# Autodesk Inventor assembly: Tensioner
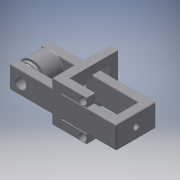
[picture p0: Inventor's stored thumbnail of the model, 180x180]
Saved by Autodesk Inventor 2017 (Build 210142000, 142)
## iProperties
Created: 2017-07-29
Part Number: Tensioner
Document SubType Name: Assembly
Designer: User
Author: User
## Documents named in this file (5)
- C:\Robotics\CAD\2016-17_CAD\DriveTrain\Tensioner.iam
- C:\Robotics\CAD\2016-17_CAD\DriveTrain\TensionerAxleHolder.ipt
- C:\Robotics\CAD\2016-17_CAD\DriveTrain\TensionerPlate.ipt
- C:\Robotics\CAD\COTSParts\Bearings - AndyMark\Bearing 250 ID 500 OD flanged_MIR.ipt
- C:\Robotics\CAD\2016-17_CAD\Custom COTS\Spacer.5inBore.378Width.ipt
## Components (5 placed, 4 different names)
1. TensionerAxleHolder:1 — Mate:1, Flush:1, Flush:2, Insert:3, Insert:4
2. TensionerPlate:1 — Mate:1, Flush:1, Flush:2
3. Bearing 250 ID 500 OD flanged_MIR:1 — Insert:3, Insert:5
4. Bearing 250 ID 500 OD flanged_MIR:2 — Insert:4
5. Spacer.5inBore.378Width:1 — Insert:5
## Relationships (6: Insert 3, Flush 2, Mate 1)
- Mate:1: TensionerAxleHolder:1 ↔ TensionerPlate:1
- Flush:1 (4.7625 mm): TensionerAxleHolder:1 ↔ TensionerPlate:1
- Flush:2 (-29.21 mm): TensionerAxleHolder:1 ↔ TensionerPlate:1
- Insert:3: TensionerAxleHolder:1 ↔ Bearing 250 ID 500 OD flanged_MIR:1
- Insert:4: TensionerAxleHolder:1 ↔ Bearing 250 ID 500 OD flanged_MIR:2
- Insert:5: Bearing 250 ID 500 OD flanged_MIR:1 ↔ Spacer.5inBore.378Width:1
